# Autodesk Inventor assembly: sborka
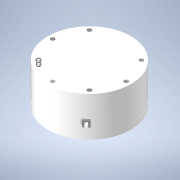
[picture p0: Inventor's stored thumbnail of the model, 180x180]
Saved by Autodesk Inventor 2020 (Build 240168000, 168)
## iProperties
Created: 2020-05-07
Part Number: sborka
Document SubType Name: Assembly
Designer: jamnissa
Mass: 192.682 g
Surface Area: 1904.41 cm^2
Volume: 119.259 cm^3
Density: 1.61565 g/cm^3
Author: jamnissa
## Documents named in this file (23)
- C:\Users\jama1\Documents\GitHub\JRobots\pcbCase\pcbCase\sborka.iam
- C:\Users\jama1\Documents\GitHub\JRobots\pcbCase\Board\PcbBoard_last3.iam
- C:\Users\jama1\Documents\GitHub\JRobots\pcbCase\motor\motor.iam
- C:\Users\jama1\Documents\GitHub\JRobots\pcbCase\wheel\Wheel.ipt
- C:\Users\jama1\Documents\GitHub\JRobots\pcbCase\soporte_plastico\soporte_plastico.ipt
- C:\Users\jama1\Documents\GitHub\JRobots\pcbCase\M3x6x25.ipt
- C:\Users\jama1\Documents\GitHub\JRobots\pcbCase\pcbCase\pcbCase_last.ipt
- C:\Users\jama1\Documents\GitHub\JRobots\pcbCase\case18650\case18650.ipt
- C:\Users\jama1\Documents\GitHub\JRobots\pcbCase\pcbCase\caseTop.ipt
- C:\Users\jama1\Documents\GitHub\JRobots\pcbCase\lidar\lidar.ipt
- C:\Users\jama1\Documents\GitHub\JRobots\pcbCase\lidar\holder.ipt
- C:\Users\jama1\Documents\GitHub\JRobots\pcbCase\pcbCase\caseBottom.ipt
- C:\Users\jama1\Documents\GitHub\JRobots\pcbCase\spacer_FF_M3x25.ipt
- C:\Users\jama1\Documents\Inventor\Content Center Files\R2020\ru-RU\Screw 2Z GOST R 50403-92\Винт A2Z.M2.5-6gx3,5 ГОСТ Р 50403-92.ipt
- C:\Users\jama1\Documents\GitHub\JRobots\pcbCase\ball\ball.iam
- C:\Users\jama1\Documents\Inventor\Content Center Files\R2020\ru-RU\Screw 2Z GOST R 50403-92\Винт A2Z.M2-6gx3 ГОСТ Р 50403-92.ipt
- C:\Users\jama1\Documents\GitHub\JRobots\pcbCase\M2.ipt
- C:\Users\jama1\Documents\Inventor\Content Center Files\R2020\ru-RU\Screw 2 GOST R 50403-92\Винт A2.M3-6gx10 ГОСТ Р 50403-92.ipt
- C:\Users\jama1\Documents\Inventor\Content Center Files\R2020\ru-RU\Screw 2Z GOST R ISO 7046-1-2013\Screw with countersunk head GOST R ISO 7046-1 - M1,6x3 - 4.8 - Z.ipt
- C:\Users\jama1\Documents\Inventor\Content Center Files\R2020\ru-RU\Screw 2Z GOST R ISO 7046-1-2013\Screw with countersunk head GOST R ISO 7046-1 - M3x10 - 4.8 - Z.ipt
- C:\Users\jama1\Documents\Inventor\Content Center Files\R2020\ru-RU\Screw 2Z GOST R ISO 7046-1-2013\Screw with countersunk head GOST R ISO 7046-1 - M3x8 - 4.8 - Z.ipt
- C:\Users\jama1\Documents\Inventor\Content Center Files\R2020\ru-RU\Screw 2 GOST R 50403-92\Винт B2.M3-6gx10 ГОСТ Р 50403-92.ipt
- C:\Users\jama1\Documents\GitHub\JRobots\pcbCase\Board\SW1.iam
## Components (61 placed, 22 different names)
1. PcbBoard_last3:1 [sub-assembly] — Совмещение:1, Совмещение:2, Совмещение:3, Совмещение:4, Вставка:26, Вставка:27, Вставка:28, Совмещение:5, Вставка:29, Вставка:30, Вставка:31, Вставка:32, Вставка:33, Вставка:36, Вставка:37, Вставка:38, Вставка:39
2. motor:1 [sub-assembly] — Совмещение:2, Вставка:2
3. motor:2 [sub-assembly] — Совмещение:1, Вставка:1
4. Wheel:1 — Вставка:1
5. Wheel:2 — Вставка:2
6. soporte_plastico:1 — Совмещение:3
7. soporte_plastico:2 — Совмещение:4
8. pcbCase_last:1 — Вставка:14, Вставка:15, Вставка:16, Вставка:18, Вставка:19, Вставка:20, Вставка:21, Вставка:24
9. case18650:1
10. M3x6x25:9 — Вставка:18
11. M3x6x25:10 — Вставка:21
12. M3x6x25:11 — Вставка:20
13. M3x6x25:12 — Вставка:19
14. M3x6x25:14 — Вставка:15
15. M3x6x25:15 — Вставка:16, Вставка:40
16. M3x6x25:16 — Вставка:14
17. caseTop:1 — Вставка:40, Совмещение:20, Совмещение:21, Совмещение:23, Совмещение:24, Совмещение:25, Совмещение:26, Совмещение:27, Совмещение:28
18. lidar:1 — Вставка:25
19. holder:1 — Вставка:24, Вставка:25
20. caseBottom:1 — Вставка:33, Совмещение:6, Совмещение:7, Совмещение:8, Совмещение:9, Совмещение:10, Совмещение:11, Совмещение:12, Совмещение:13, Вставка:34, Вставка:35, Совмещение:14, Совмещение:15, Совмещение:16, Совмещение:17
21. spacer_FF_M3x25:1 — Вставка:31
22. spacer_FF_M3x25:2 — Вставка:32
23. spacer_FF_M3x25:3 — Вставка:30
24. spacer_FF_M3x25:4 — Вставка:26
25. spacer_FF_M3x25:5 — Вставка:29
26. spacer_FF_M3x25:6 — Совмещение:5
27. spacer_FF_M3x25:7 — Вставка:27
28. spacer_FF_M3x25:8 — Вставка:28
29. Винт 2Z ГОСТ Р 50403-92 M2.5x3,5-A:1 — Совмещение:6
30. Винт 2Z ГОСТ Р 50403-92 M2.5x3,5-A:2 — Совмещение:7
31. Винт 2Z ГОСТ Р 50403-92 M2.5x3,5-A:3 — Совмещение:8
32. Винт 2Z ГОСТ Р 50403-92 M2.5x3,5-A:4 — Совмещение:9
33. Винт 2Z ГОСТ Р 50403-92 M2.5x3,5-A:5 — Совмещение:10, Совмещение:19
34. Винт 2Z ГОСТ Р 50403-92 M2.5x3,5-A:6 — Совмещение:11
35. Винт 2Z ГОСТ Р 50403-92 M2.5x3,5-A:7 — Совмещение:12
36. Винт 2Z ГОСТ Р 50403-92 M2.5x3,5-A:8 — Совмещение:13
37. ball:1 [sub-assembly] — Вставка:35
38. ball:2 [sub-assembly] — Вставка:34
39. Винт 2Z ГОСТ Р 50403-92 M2x3-A:1 — Совмещение:14
40. Винт 2Z ГОСТ Р 50403-92 M2x3-A:2 — Совмещение:15
41. Винт 2Z ГОСТ Р 50403-92 M2x3-A:3 — Совмещение:16
42. Винт 2Z ГОСТ Р 50403-92 M2x3-A:4 — Совмещение:17
43. M2:1 — Вставка:36
44. M2:2 — Вставка:37
45. M2:3 — Вставка:39
46. M2:4 — Вставка:38
47. ISO 7046-1 Z c M1,6 x 3 - 4.8 - Z:1 — Совмещение:19
48. ISO 7046-1 Z c M3 x 10 - 4.8 - Z:1
49. ISO 7046-1 Z c M3 x 10 - 4.8 - Z:2
50. ISO 7046-1 Z c M3 x 10 - 4.8 - Z:3
51. ISO 7046-1 Z c M3 x 10 - 4.8 - Z:4
52. ISO 7046-1 Z c M3 x 10 - 4.8 - Z:5
53. ISO 7046-1 Z c M3 x 8 - 4.8 - Z:1
54. Винт 2 ГОСТ Р 50403-92 M3x10-A:2 — Совмещение:20
55. Винт 2 ГОСТ Р 50403-92 M3x10-A:3 — Совмещение:21
56. Винт 2 ГОСТ Р 50403-92 M3x10-B:1 — Совмещение:23
57. Винт 2 ГОСТ Р 50403-92 M3x10-B:2 — Совмещение:24
58. Винт 2 ГОСТ Р 50403-92 M3x10-B:3 — Совмещение:25
59. Винт 2 ГОСТ Р 50403-92 M3x10-B:4 — Совмещение:26
60. Винт 2 ГОСТ Р 50403-92 M3x10-B:5 — Совмещение:27
61. SW1:1 [sub-assembly] — Совмещение:28
## Relationships (52: Mate 26, Insert 26)
- Совмещение:1 [Mate]: PcbBoard_last3:1 ↔ motor:2
- Совмещение:2 [Mate]: PcbBoard_last3:1 ↔ motor:1
- Вставка:1 [Insert] (1 mm): motor:2 ↔ Wheel:1
- Вставка:2 [Insert] (1 mm): motor:1 ↔ Wheel:2
- Совмещение:3 [Mate]: PcbBoard_last3:1 ↔ soporte_plastico:1
- Совмещение:4 [Mate]: PcbBoard_last3:1 ↔ soporte_plastico:2
- Вставка:14 [Insert]: pcbCase_last:1 ↔ M3x6x25:16
- Вставка:15 [Insert]: pcbCase_last:1 ↔ M3x6x25:14
- Вставка:16 [Insert]: pcbCase_last:1 ↔ M3x6x25:15
- Вставка:18 [Insert]: pcbCase_last:1 ↔ M3x6x25:9
- Вставка:19 [Insert]: pcbCase_last:1 ↔ M3x6x25:12
- Вставка:20 [Insert]: pcbCase_last:1 ↔ M3x6x25:11
- Вставка:21 [Insert]: pcbCase_last:1 ↔ M3x6x25:10
- Вставка:24 [Insert] (-2 mm): pcbCase_last:1 ↔ holder:1
- Вставка:25 [Insert]: lidar:1 ↔ holder:1
- Вставка:26 [Insert]: PcbBoard_last3:1 ↔ spacer_FF_M3x25:4
- Вставка:27 [Insert]: PcbBoard_last3:1 ↔ spacer_FF_M3x25:7
- Вставка:28 [Insert]: PcbBoard_last3:1 ↔ spacer_FF_M3x25:8
- Совмещение:5 [Mate]: PcbBoard_last3:1 ↔ spacer_FF_M3x25:6
- Вставка:29 [Insert]: PcbBoard_last3:1 ↔ spacer_FF_M3x25:5
- Вставка:30 [Insert]: PcbBoard_last3:1 ↔ spacer_FF_M3x25:3
- Вставка:31 [Insert]: PcbBoard_last3:1 ↔ spacer_FF_M3x25:1
- Вставка:32 [Insert]: PcbBoard_last3:1 ↔ spacer_FF_M3x25:2
- Вставка:33 [Insert]: PcbBoard_last3:1 ↔ caseBottom:1
- Совмещение:6 [Mate]: caseBottom:1 ↔ Винт 2Z ГОСТ Р 50403-92 M2.5x3,5-A:1
- Совмещение:7 [Mate]: caseBottom:1 ↔ Винт 2Z ГОСТ Р 50403-92 M2.5x3,5-A:2
- Совмещение:8 [Mate]: caseBottom:1 ↔ Винт 2Z ГОСТ Р 50403-92 M2.5x3,5-A:3
- Совмещение:9 [Mate]: caseBottom:1 ↔ Винт 2Z ГОСТ Р 50403-92 M2.5x3,5-A:4
- Совмещение:10 [Mate]: caseBottom:1 ↔ Винт 2Z ГОСТ Р 50403-92 M2.5x3,5-A:5
- Совмещение:11 [Mate]: caseBottom:1 ↔ Винт 2Z ГОСТ Р 50403-92 M2.5x3,5-A:6
- Совмещение:12 [Mate]: caseBottom:1 ↔ Винт 2Z ГОСТ Р 50403-92 M2.5x3,5-A:7
- Совмещение:13 [Mate]: caseBottom:1 ↔ Винт 2Z ГОСТ Р 50403-92 M2.5x3,5-A:8
- Вставка:34 [Insert]: caseBottom:1 ↔ ball:2
- Вставка:35 [Insert]: caseBottom:1 ↔ ball:1
- Совмещение:14 [Mate]: caseBottom:1 ↔ Винт 2Z ГОСТ Р 50403-92 M2x3-A:1
- Совмещение:15 [Mate]: caseBottom:1 ↔ Винт 2Z ГОСТ Р 50403-92 M2x3-A:2
- Совмещение:16 [Mate]: caseBottom:1 ↔ Винт 2Z ГОСТ Р 50403-92 M2x3-A:3
- Совмещение:17 [Mate]: caseBottom:1 ↔ Винт 2Z ГОСТ Р 50403-92 M2x3-A:4
- Вставка:36 [Insert]: PcbBoard_last3:1 ↔ M2:1
- Вставка:37 [Insert]: PcbBoard_last3:1 ↔ M2:2
- Вставка:38 [Insert]: PcbBoard_last3:1 ↔ M2:4
- Вставка:39 [Insert]: PcbBoard_last3:1 ↔ M2:3
- Вставка:40 [Insert]: M3x6x25:15 ↔ caseTop:1
- Совмещение:19 [Mate]: Винт 2Z ГОСТ Р 50403-92 M2.5x3,5-A:5 ↔ ISO 7046-1 Z c M1,6 x 3 - 4.8 - Z:1
- Совмещение:20 [Mate]: caseTop:1 ↔ Винт 2 ГОСТ Р 50403-92 M3x10-A:2
- Совмещение:21 [Mate]: caseTop:1 ↔ Винт 2 ГОСТ Р 50403-92 M3x10-A:3
- Совмещение:23 [Mate]: caseTop:1 ↔ Винт 2 ГОСТ Р 50403-92 M3x10-B:1
- Совмещение:24 [Mate]: caseTop:1 ↔ Винт 2 ГОСТ Р 50403-92 M3x10-B:2
- Совмещение:25 [Mate]: caseTop:1 ↔ Винт 2 ГОСТ Р 50403-92 M3x10-B:3
- Совмещение:26 [Mate]: caseTop:1 ↔ Винт 2 ГОСТ Р 50403-92 M3x10-B:4
- Совмещение:27 [Mate]: caseTop:1 ↔ Винт 2 ГОСТ Р 50403-92 M3x10-B:5
- Совмещение:28 [Mate]: caseTop:1 ↔ SW1:1
